# Autodesk Inventor assembly: HB8_920.1-sunhub8_casing_top
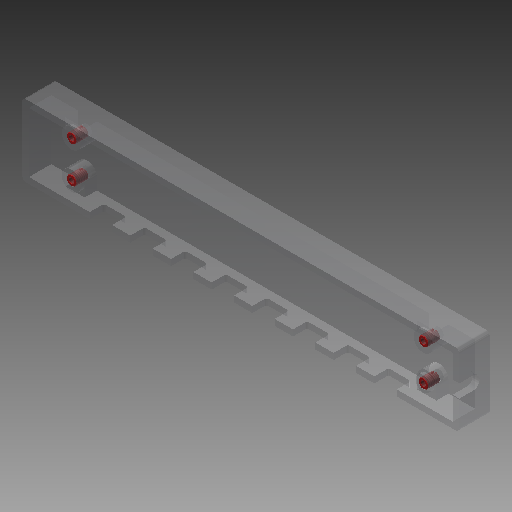
[picture p0: Inventor's stored thumbnail of the model, 512x512]
Saved by Autodesk Inventor 2019 (Build 230136000, 136)
## iProperties
Created: 2019-03-01
Part Number: HB8_920.1-sunhub8_casing_top
Document SubType Name: Assembly
Designer: Rene
Author: Rene
## Documents named in this file (3)
- C:\dev\c-scape\hardponics\dwg\sunhub\HB8_920.1-sunhub8_casing_top.iam
- C:\dev\c-scape\hardponics\dwg\sunhub\SH8_002.1-sunhub8-casing_top.ipt
- C:\dev\c-scape\hardponics\dwg\sunhub\XGEN_M3_draadbus_4x6mm.ipt
## Components (5 placed, 2 different names)
1. SH8_002.1-sunhub8-casing_top:1 — Insert:1, Insert:2, Insert:3, Insert:4
2. XGEN_M3_draadbus_4x6mm:1 — Insert:1
3. XGEN_M3_draadbus_4x6mm:2 — Insert:2
4. XGEN_M3_draadbus_4x6mm:3 — Insert:4
5. XGEN_M3_draadbus_4x6mm:4 — Insert:3
## Relationships (4: Insert 4)
- Insert:1: SH8_002.1-sunhub8-casing_top:1 ↔ XGEN_M3_draadbus_4x6mm:1
- Insert:2: SH8_002.1-sunhub8-casing_top:1 ↔ XGEN_M3_draadbus_4x6mm:2
- Insert:3: SH8_002.1-sunhub8-casing_top:1 ↔ XGEN_M3_draadbus_4x6mm:4
- Insert:4: SH8_002.1-sunhub8-casing_top:1 ↔ XGEN_M3_draadbus_4x6mm:3
